# Autodesk Inventor assembly: motor_channel_mirrored
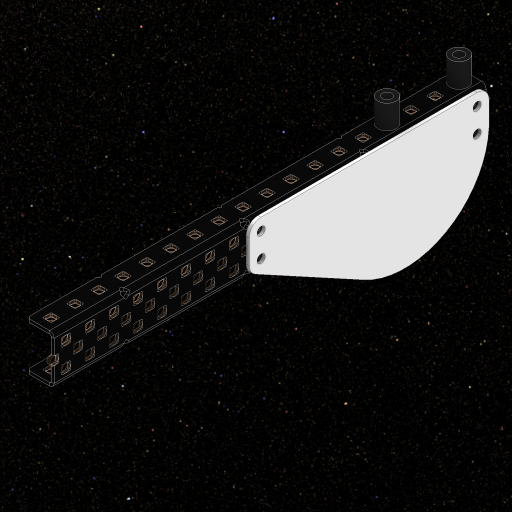
[picture p0: Inventor's stored thumbnail of the model, 512x512]
Saved by Autodesk Inventor 2024 (Build 280153000, 153)
## iProperties
Created: 2024-02-22
Part Number: motor_channel_mirrored
Document SubType Name: Assembly
Designer: Averey Ku
Author: Averey Ku
## Documents named in this file (8)
- D:\vex_robotics\hardware\cad\lil_zoom\intake\mirrored_parts\motor_channel_mirrored.iam
- D:\vex_robotics\hardware\cad\lil_zoom\intake\mirrored_parts\Alu C 1x2x1x18_mirrored.ipt
- D:\vex_robotics\hardware\cad\lil_zoom\intake\mirrored_parts\HS Bearing Flat_mirrored.ipt
- D:\vex_robotics\hardware\cad\lil_zoom\intake\mirrored_parts\intake_sled_mirrored.ipt
- D:\vex_robotics\hardware\cad\VEX-CAD-Inventor-1.41\Motion\Spacers\Spacer Nylon .375 OD\NSpacer .375 OD x .500.ipt
- D:\vex_robotics\hardware\cad\VEX-CAD-Inventor-1.41\Motion\Spacers\Spacer Nylon .375 OD.ipt
- D:\vex_robotics\hardware\cad\VEX-CAD-Inventor-1.41\Structure\Standoff\Standoff .875.ipt
- D:\vex_robotics\hardware\cad\VEX-CAD-Inventor-1.41\Structure\Standoff.ipt
## Components (7 placed, 5 different names)
1. Alu C 1x2x1x18_mirrored:1 — Mate:1, Insert:5, Insert:13, Insert:14, Insert:16, Insert:17, Insert:18, Mate:2
2. HS Bearing Flat_mirrored:1 — Mate:1, Insert:5
3. intake_sled_mirrored:1 — Insert:18, Mate:2
4. NSpacer .375 OD x .500:1 — Insert:13
5. NSpacer .375 OD x .500:2 — Insert:14
6. Standoff .875:1 — Insert:16
7. Standoff .875:2 — Insert:17
## Relationships (8: Insert 6, Mate 2)
- Mate:1: Alu C 1x2x1x18_mirrored:1 ↔ HS Bearing Flat_mirrored:1
- Insert:5: Alu C 1x2x1x18_mirrored:1 ↔ HS Bearing Flat_mirrored:1
- Insert:13: Alu C 1x2x1x18_mirrored:1 ↔ NSpacer .375 OD x .500:1
- Insert:14: Alu C 1x2x1x18_mirrored:1 ↔ NSpacer .375 OD x .500:2
- Insert:16: Alu C 1x2x1x18_mirrored:1 ↔ Standoff .875:1
- Insert:17: Alu C 1x2x1x18_mirrored:1 ↔ Standoff .875:2
- Insert:18: Alu C 1x2x1x18_mirrored:1 ↔ intake_sled_mirrored:1
- Mate:2: Alu C 1x2x1x18_mirrored:1 ↔ intake_sled_mirrored:1
